# Autodesk Inventor assembly: center wheel assembly
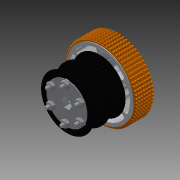
[picture p0: Inventor's stored thumbnail of the model, 180x180]
Saved by Autodesk Inventor 2014 SP1 (Build 180222100, 222)
## iProperties
Created: 2014-01-05
Part Number: center wheel assembly
Document SubType Name: Assembly
Designer: Arpan
Mass: 388.119 g
Surface Area: 1257.09 cm^2
Volume: 187.127 cm^3
Density: 2.07409 g/cm^3
Author: Arpan
## Documents named in this file (7)
- C:\Users\Arpan\Documents\GitHub\2014buildCAD\chassisdrivetrain\chassis light\COTS items\center wheel assembly.iam
- C:\Users\Arpan\Documents\GitHub\2014buildCAD\chassisdrivetrain\chassis light\COTS items\4 Inch Performance Wheel Tread.ipt
- C:\Users\Arpan\Documents\GitHub\2014buildCAD\chassisdrivetrain\chassis light\COTS items\4 Perf ThruTread 500 Hex (1).ipt
- C:\Users\Arpan\Documents\GitHub\2014buildCAD\chassisdrivetrain\chassis light\COTS items\DBK_42ToothPulley V2.iam
- C:\Users\Arpan\Documents\GitHub\2014buildCAD\chassisdrivetrain\chassis light\500_hex_hub.ipt
- C:\Users\Arpan\Documents\GitHub\2014buildCAD\hardware\10-24\3 inch screw 91251A084.ipt
- C:\Users\Arpan\Documents\GitHub\2014buildCAD\hardware\10-24\thin hex locknut 90633A011.ipt
## Components (17 placed, 6 different names)
1. 4 Inch Performance Wheel Tread:1 — Mate:1, Mate:2
2. 4 Perf ThruTread 500 Hex (1):1 — Mate:1, Mate:2, Mate:22, Mate:23, Mate:24, Mate:25, Mate:26, Mate:27, Mate:28, Mate:29, Mate:30, Mate:31, Mate:32, Mate:33
3. DBK_42ToothPulley V2:2 [sub-assembly]
4. DBK_42ToothPulley V2:3 [sub-assembly] — Mate:21
5. 500_hex_hub:1 — Mate:21, Mate:35, Mate:36, Mate:38, Mate:40, Mate:42, Mate:44
6. 3 inch screw 91251A084:1 — Mate:25, Mate:28, Mate:37
7. 3 inch screw 91251A084:2 — Mate:24, Mate:29, Mate:39
8. 3 inch screw 91251A084:3 — Mate:23, Mate:30, Mate:41
9. 3 inch screw 91251A084:4 — Mate:22, Mate:31, Mate:43
10. 3 inch screw 91251A084:5 — Mate:27, Mate:32, Mate:45
11. 3 inch screw 91251A084:6 — Mate:26, Mate:33, Mate:34
12. thin hex locknut 90633A011:1 — Mate:34, Mate:35
13. thin hex locknut 90633A011:2 — Mate:38, Mate:39
14. thin hex locknut 90633A011:3 — Mate:40, Mate:41
15. thin hex locknut 90633A011:4 — Mate:44, Mate:45
16. thin hex locknut 90633A011:5 — Mate:42, Mate:43
17. thin hex locknut 90633A011:6 — Mate:36, Mate:37
## Relationships (27: Mate 27)
- Mate:1: 4 Inch Performance Wheel Tread:1 ↔ 4 Perf ThruTread 500 Hex (1):1
- Mate:2: 4 Inch Performance Wheel Tread:1 ↔ 4 Perf ThruTread 500 Hex (1):1
- Mate:21: DBK_42ToothPulley V2:3 ↔ 500_hex_hub:1
- Mate:22: 4 Perf ThruTread 500 Hex (1):1 ↔ 3 inch screw 91251A084:4
- Mate:23: 4 Perf ThruTread 500 Hex (1):1 ↔ 3 inch screw 91251A084:3
- Mate:24: 4 Perf ThruTread 500 Hex (1):1 ↔ 3 inch screw 91251A084:2
- Mate:25: 4 Perf ThruTread 500 Hex (1):1 ↔ 3 inch screw 91251A084:1
- Mate:26: 4 Perf ThruTread 500 Hex (1):1 ↔ 3 inch screw 91251A084:6
- Mate:27: 4 Perf ThruTread 500 Hex (1):1 ↔ 3 inch screw 91251A084:5
- Mate:28: 4 Perf ThruTread 500 Hex (1):1 ↔ 3 inch screw 91251A084:1
- Mate:29: 4 Perf ThruTread 500 Hex (1):1 ↔ 3 inch screw 91251A084:2
- Mate:30: 4 Perf ThruTread 500 Hex (1):1 ↔ 3 inch screw 91251A084:3
- Mate:31: 4 Perf ThruTread 500 Hex (1):1 ↔ 3 inch screw 91251A084:4
- Mate:32: 4 Perf ThruTread 500 Hex (1):1 ↔ 3 inch screw 91251A084:5
- Mate:33: 4 Perf ThruTread 500 Hex (1):1 ↔ 3 inch screw 91251A084:6
- Mate:34: 3 inch screw 91251A084:6 ↔ thin hex locknut 90633A011:1
- Mate:35: 500_hex_hub:1 ↔ thin hex locknut 90633A011:1
- Mate:36: 500_hex_hub:1 ↔ thin hex locknut 90633A011:6
- Mate:37: 3 inch screw 91251A084:1 ↔ thin hex locknut 90633A011:6
- Mate:38: 500_hex_hub:1 ↔ thin hex locknut 90633A011:2
- Mate:39: 3 inch screw 91251A084:2 ↔ thin hex locknut 90633A011:2
- Mate:40: 500_hex_hub:1 ↔ thin hex locknut 90633A011:3
- Mate:41: 3 inch screw 91251A084:3 ↔ thin hex locknut 90633A011:3
- Mate:42: 500_hex_hub:1 ↔ thin hex locknut 90633A011:5
- Mate:43: 3 inch screw 91251A084:4 ↔ thin hex locknut 90633A011:5
- Mate:44: 500_hex_hub:1 ↔ thin hex locknut 90633A011:4
- Mate:45: 3 inch screw 91251A084:5 ↔ thin hex locknut 90633A011:4
